# Autodesk Inventor assembly: Assembly1
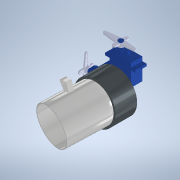
[picture p0: Inventor's stored thumbnail of the model, 180x180]
Saved by Autodesk Inventor 2021 (Build 250183000, 183)
## iProperties
Created: 2021-07-19
Part Number: Assembly1
Document SubType Name: Assembly
Designer: samlo
Author: samlo
## Documents named in this file (5)
- C:\Users\samlo\OneDrive\Documents\Assembly1.iam
- C:\Users\samlo\OneDrive\Documents\top tvc.ipt
- C:\Users\samlo\OneDrive\Documents\bottom tvc.ipt
- C:\Users\samlo\Downloads\servo-motor-sg90-7.snapshot.4\servorough_body.ipt
- C:\Users\samlo\Downloads\tower-pro-micro-servo-sg90-horn-1.snapshot.2\Tower pro micro servo SG90 HORN.ipt
## Components (6 placed, 4 different names)
1. top tvc:1 — Ball:1, Mate:2, Mate:3, Tangent:1
2. bottom tvc:1 — Ball:1
3. servorough_body:1 — Mate:2, Mate:5
4. servorough_body:2 — Mate:3, Tangent:1, Angle:1, Mate:4
5. Tower pro micro servo SG90 HORN:1 — Mate:5
6. Tower pro micro servo SG90 HORN:2 — Angle:1, Mate:4
## Relationships (7: Mate 4, BallJoint 1, Tangent 1, Angle 1)
- Ball:1: top tvc:1 ↔ bottom tvc:1
- Mate:2: top tvc:1 ↔ servorough_body:1
- Mate:3: top tvc:1 ↔ servorough_body:2
- Tangent:1: top tvc:1 ↔ servorough_body:2
- Angle:1 (0 deg): servorough_body:2 ↔ Tower pro micro servo SG90 HORN:2
- Mate:4: servorough_body:2 ↔ Tower pro micro servo SG90 HORN:2
- Mate:5: servorough_body:1 ↔ Tower pro micro servo SG90 HORN:1
